# Autodesk Inventor assembly: Assembly1
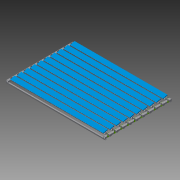
[picture p0: Inventor's stored thumbnail of the model, 180x180]
Saved by Autodesk Inventor 2015 SP1 (Build 190203100, 203)
## iProperties
Created: 2015-03-28
Part Number: Assembly1
Document SubType Name: Assembly
Designer: Cyril
Mass: 10678.5 g
Surface Area: 59183.2 cm^2
Volume: 10678.5 cm^3
Density: 1 g/cm^3
Author: Cyril
## Documents named in this file (10)
- C:\Users\Cyril\Documents\OSE FR\Concentrateur solaire\Inventor\Assemblage_cadre-miroir.iam
- C:\Users\Cyril\Documents\OSE FR\Concentrateur solaire\Inventor\Part4.ipt
- C:\Users\Cyril\Documents\OSE FR\Concentrateur solaire\Inventor\Assemblage_miroir.iam
- C:\Users\Cyril\Documents\OSE FR\Concentrateur solaire\Inventor\Moteur.ipt
- C:\Users\Cyril\Documents\OSE FR\Concentrateur solaire\Inventor\Accouplement.ipt
- C:\Users\Cyril\Documents\OSE FR\Concentrateur solaire\Inventor\michaud_chailly_C2_151_8_128.ipt
- C:\Users\Cyril\Documents\OSE FR\Concentrateur solaire\Inventor\Plaque support_D.ipt
- C:\Users\Cyril\Documents\OSE FR\Concentrateur solaire\Inventor\Assemblage_Cadre.iam
- C:\Users\Cyril\Documents\OSE FR\Concentrateur solaire\Inventor\Capteur optique.ipt
- C:\Users\Cyril\Documents\OSE FR\Concentrateur solaire\Inventor\Plaque support_G.ipt
## Components (91 placed, 9 different names)
1. Assemblage_Cadre:1 [sub-assembly] — Insert:37, Flush:34, Flush:35, Flush:36, Insert:38, Insert:39, Insert:40, Insert:41, Insert:43
2. Moteur:1 — Insert:19, Insert:23, Insert:24
3. Part4:1 — Insert:23, Insert:24, Insert:37, Insert:38
4. Plaque support_D:1 — Insert:21, Insert:25, Mate:4, Insert:39, Insert:43
5. Assemblage_miroir:3 [sub-assembly] — Insert:20, Mate:3
6. michaud_chailly_C2_151_8_128:1 — Insert:21, Mate:3
7. Accouplement:1 — Insert:19, Insert:20
8. Capteur optique:1 — Insert:25, Mate:4
9. Plaque support_G:1 — Insert:40, Insert:41, Insert:42
10. michaud_chailly_C2_151_8_128:11 — Insert:42
11. Moteur:2
12. Part4:2
13. Plaque support_D:3
14. Assemblage_miroir:4 [sub-assembly]
15. michaud_chailly_C2_151_8_128:2
16. Accouplement:2
17. Capteur optique:2
18. Plaque support_G:2
19. michaud_chailly_C2_151_8_128:12
20. Moteur:3
21. Part4:3
22. Plaque support_D:4
23. Assemblage_miroir:5 [sub-assembly]
24. michaud_chailly_C2_151_8_128:3
25. Accouplement:3
26. Capteur optique:3
27. Plaque support_G:3
28. michaud_chailly_C2_151_8_128:13
29. Moteur:4
30. Part4:4
31. Plaque support_D:5
32. Assemblage_miroir:6 [sub-assembly]
33. michaud_chailly_C2_151_8_128:4
34. Accouplement:4
35. Capteur optique:4
36. Plaque support_G:4
37. michaud_chailly_C2_151_8_128:14
38. Moteur:5
39. Part4:5
40. Plaque support_D:6
41. Assemblage_miroir:7 [sub-assembly]
42. michaud_chailly_C2_151_8_128:5
43. Accouplement:5
44. Capteur optique:5
45. Plaque support_G:5
46. michaud_chailly_C2_151_8_128:15
47. Moteur:6
48. Part4:6
49. Plaque support_D:7
50. Assemblage_miroir:8 [sub-assembly]
51. michaud_chailly_C2_151_8_128:6
52. Accouplement:6
53. Capteur optique:6
54. Plaque support_G:6
55. michaud_chailly_C2_151_8_128:16
56. Moteur:7
57. Part4:7
58. Plaque support_D:8
59. Assemblage_miroir:9 [sub-assembly]
60. michaud_chailly_C2_151_8_128:7
61. Accouplement:7
62. Capteur optique:7
63. Plaque support_G:7
64. michaud_chailly_C2_151_8_128:17
65. Moteur:8
66. Part4:8
67. Plaque support_D:9
68. Assemblage_miroir:10 [sub-assembly]
69. michaud_chailly_C2_151_8_128:8
70. Accouplement:8
71. Capteur optique:8
72. Plaque support_G:8
73. michaud_chailly_C2_151_8_128:18
74. Moteur:9
75. Part4:9
76. Plaque support_D:10
77. Assemblage_miroir:11 [sub-assembly]
78. michaud_chailly_C2_151_8_128:9
79. Accouplement:9
80. Capteur optique:9
81. Plaque support_G:9
82. michaud_chailly_C2_151_8_128:19
83. Moteur:10
84. Part4:10
85. Plaque support_D:11
86. Assemblage_miroir:12 [sub-assembly]
87. michaud_chailly_C2_151_8_128:10
88. Accouplement:10
89. Capteur optique:10
90. Plaque support_G:10
91. michaud_chailly_C2_151_8_128:20
## Component patterns: (10 elements, first: Moteur:1 + Part4:1 + Plaque support_D:1 + Assemblage_miroir:3 + michaud_chailly_C2_151_8_128:1 + Accouplement:1 + Capteur optique:1 + Plaque support_G:1 + michaud_chailly_C2_151_8_128:11)
## Relationships (18: Insert 13, Flush 3, Mate 2)
- Insert:19 (-10 mm): Moteur:1 ↔ Accouplement:1
- Insert:20 (-8 mm): Assemblage_miroir:3 ↔ Accouplement:1
- Insert:21: Plaque support_D:1 ↔ michaud_chailly_C2_151_8_128:1
- Insert:23: Moteur:1 ↔ Part4:1
- Insert:24: Moteur:1 ↔ Part4:1
- Mate:3: Assemblage_miroir:3 ↔ michaud_chailly_C2_151_8_128:1
- Insert:25: Plaque support_D:1 ↔ Capteur optique:1
- Mate:4: Plaque support_D:1 ↔ Capteur optique:1
- Insert:37: Assemblage_Cadre:1 ↔ Part4:1
- Flush:34: Assemblage_Cadre:1
- Flush:35: Assemblage_Cadre:1
- Flush:36: Assemblage_Cadre:1
- Insert:38: Assemblage_Cadre:1 ↔ Part4:1
- Insert:39: Assemblage_Cadre:1 ↔ Plaque support_D:1
- Insert:40: Assemblage_Cadre:1 ↔ Plaque support_G:1
- Insert:41: Assemblage_Cadre:1 ↔ Plaque support_G:1
- Insert:42: Plaque support_G:1 ↔ michaud_chailly_C2_151_8_128:11
- Insert:43: Assemblage_Cadre:1 ↔ Plaque support_D:1
